# Autodesk Inventor assembly: Engine Assembly
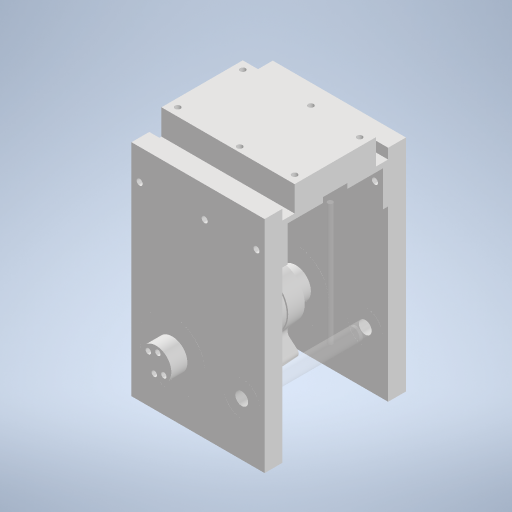
[picture p0: Inventor's stored thumbnail of the model, 512x512]
Saved by Autodesk Inventor 2023 (Build 270158000, 158)
## iProperties
Created: 2022-12-22
Part Number: Engine Assembly
Document SubType Name: Assembly
Designer: tgr41
Author: tgr41
## Documents named in this file (7)
- C:\Users\tgr41\OneDrive\Documents\Repositories\Steam-Engine\2 Inch V3\Engine Assembly.iam
- C:\Users\tgr41\OneDrive\Documents\Repositories\Steam-Engine\2 Inch V3\Piston Subassembly.iam
- C:\Users\tgr41\OneDrive\Documents\Repositories\Steam-Engine\2 Inch V3\Connecting Rod.iam
- C:\Users\tgr41\OneDrive\Documents\Repositories\Steam-Engine\2 Inch V3\Head Cylinder and Frame Subassembly.iam
- C:\Users\tgr41\OneDrive\Documents\Repositories\Steam-Engine\2 Inch V3\Crankshaft Subassembly.iam
- C:\Users\tgr41\OneDrive\Documents\Repositories\Steam-Engine\2 Inch V3\Cam Shaft Test.ipt
- C:\Users\tgr41\OneDrive\Documents\Repositories\Steam-Engine\2 Inch V3\Valve Test.ipt
## Components (7 placed, 6 different names)
1. Piston Subassembly:1 [sub-assembly] — Mate:1, Mate:2, Mate:3, Flush:1
2. Connecting Rod:1 [sub-assembly] — Mate:1, Mate:2, Mate:4, Mate:5, Mate:6, Mate:7
3. Head Cylinder and Frame Subassembly:1 [sub-assembly] — Mate:3, Angle:1, Flush:1, Mate:14, Flush:2, Mate:15
4. Crankshaft Subassembly:1 [sub-assembly] — Mate:6, Mate:7, Angle:1, Mate:8
5. Crankshaft Subassembly:2 [sub-assembly] — Mate:4, Mate:5, Mate:8
6. Cam Shaft Test:1 — Mate:14, Flush:2, Mate:16
7. Valve Test:1 — Mate:15, Mate:16
## Relationships (14: Mate 11, Flush 2, Angle 1)
- Mate:1: Piston Subassembly:1 ↔ Connecting Rod:1
- Mate:2: Piston Subassembly:1 ↔ Connecting Rod:1
- Mate:3: Piston Subassembly:1 ↔ Head Cylinder and Frame Subassembly:1
- Mate:4: Connecting Rod:1 ↔ Crankshaft Subassembly:2
- Mate:5: Connecting Rod:1 ↔ Crankshaft Subassembly:2
- Mate:6: Connecting Rod:1 ↔ Crankshaft Subassembly:1
- Mate:7: Connecting Rod:1 ↔ Crankshaft Subassembly:1
- Angle:1 (0 deg): Head Cylinder and Frame Subassembly:1 ↔ Crankshaft Subassembly:1
- Mate:8: Crankshaft Subassembly:1 ↔ Crankshaft Subassembly:2
- Flush:1: Piston Subassembly:1 ↔ Head Cylinder and Frame Subassembly:1
- Mate:14: Head Cylinder and Frame Subassembly:1 ↔ Cam Shaft Test:1
- Flush:2: Head Cylinder and Frame Subassembly:1 ↔ Cam Shaft Test:1
- Mate:15: Head Cylinder and Frame Subassembly:1 ↔ Valve Test:1
- Mate:16: Cam Shaft Test:1 ↔ Valve Test:1
